# Autodesk Inventor assembly: 150-6-200 (50N) Gas Spring
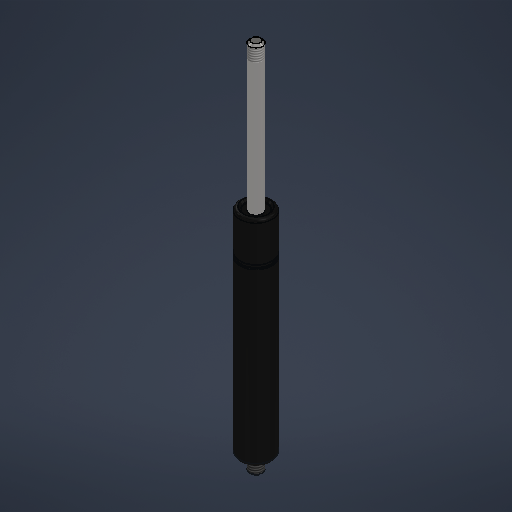
[picture p0: Inventor's stored thumbnail of the model, 512x512]
Saved by Autodesk Inventor 2026 (Build 300175050, 175E)
## iProperties
Created: 2025-07-03
Part Number: 150-6-200 (50N) Gas Spring
Document SubType Name: Assembly
Designer: Joshua Eah
Author: Joshua Eah
## Documents named in this file (3)
- C:\Users\Joshua Eah\Documents\GitHub\Voron-0\CAD\Master Assembly\Extras\Gas Spring\150-6-200 (50N) Gas Spring.iam
- C:\Users\Joshua Eah\Documents\GitHub\Voron-0\CAD\Master Assembly\Extras\Gas Spring\Rod.ipt
- C:\Users\Joshua Eah\Documents\GitHub\Voron-0\CAD\Master Assembly\Extras\Gas Spring\Cylinder.ipt
## Components (2 placed, 2 different names)
1. Cylinder:1 — Cylindrical:1
2. Rod:1 — Cylindrical:1
## Relationships (1: CylindricalJoint 1)
- Cylindrical:1: Cylinder:1 ↔ Rod:1
